# Autodesk Inventor assembly: EXTRUDER
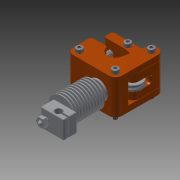
[picture p0: Inventor's stored thumbnail of the model, 180x180]
Saved by Autodesk Inventor 2013 (Build 170138000, 138)
## iProperties
Created: 2014-06-22
Part Number: EXTRUDER
Document SubType Name: Assembly
Designer: employee
Author: employee
## Documents named in this file (12)
- C:\Users\employee\Desktop\CoreXZ 2\EXTRUDER.iam
- C:\Users\employee\Desktop\CoreXZ 2\EXTRUDER BODY.ipt
- C:\Users\employee\Desktop\CoreXZ 2\E3Dv6.ipt
- C:\Users\employee\Desktop\CoreXZ 2\EXTRUDER BODY_MIR.ipt
- C:\Users\employee\Desktop\CoreXZ 2\EXTRUDER ARM.ipt
- C:\Users\employee\Desktop\CoreXZ 2\HOBBED PULLEY.ipt
- C:\Users\employee\Desktop\CoreXZ 2\625vv.ipt
- C:\Users\employee\Desktop\CoreXZ 2\EXTRUDER ARM_MIR.ipt
- C:\Users\employee\Desktop\CoreXZ 2\EXTRUDER SPRING.ipt
- C:\Users\employee\Desktop\CoreXZ 2\M3 SQUARE NUT.ipt
- C:\Users\employee\Desktop\CoreXZ 2\M3X35.ipt
- C:\Users\employee\Desktop\CoreXZ 2\M3X20.ipt
## Components (14 placed, 11 different names)
1. EXTRUDER BODY:1 — Insert:1, Angle:1, Flush:2, Insert:4, Angle:2, Insert:9
2. E3Dv6:1 — Insert:1, Angle:1
3. EXTRUDER BODY_MIR:1 — Mate:1, Insert:6, Insert:7, Insert:8
4. EXTRUDER ARM:1 — Insert:2, Insert:3, Flush:3, Insert:4, Mate:2, Flush:4
5. HOBBED PULLEY:1 — Mate:1, Flush:2
6. 625vv:1 — Insert:2
7. EXTRUDER ARM_MIR:1 — Insert:3, Flush:3, Insert:10
8. EXTRUDER SPRING:1 — Mate:2, Flush:4, Tangent:1, Mate:3, Mate:4
9. M3 SQUARE NUT:1 — Angle:2, Tangent:1, Mate:3
10. M3X35:1 — Insert:6
11. M3X35:2 — Insert:7
12. M3X35:3 — Insert:8
13. M3X35:4 — Insert:9, Mate:4
14. M3X20:1 — Insert:10
## Relationships (19: Insert 9, Mate 4, Flush 3, Angle 2, Tangent 1)
- Insert:1: EXTRUDER BODY:1 ↔ E3Dv6:1
- Angle:1 (0 deg): EXTRUDER BODY:1 ↔ E3Dv6:1
- Mate:1: EXTRUDER BODY_MIR:1 ↔ HOBBED PULLEY:1
- Flush:2 (7.38 mm): EXTRUDER BODY:1 ↔ HOBBED PULLEY:1
- Insert:2: EXTRUDER ARM:1 ↔ 625vv:1
- Insert:3: EXTRUDER ARM:1 ↔ EXTRUDER ARM_MIR:1
- Flush:3: EXTRUDER ARM:1 ↔ EXTRUDER ARM_MIR:1
- Insert:4: EXTRUDER BODY:1 ↔ EXTRUDER ARM:1
- Mate:2: EXTRUDER ARM:1 ↔ EXTRUDER SPRING:1
- Flush:4: EXTRUDER ARM:1 ↔ EXTRUDER SPRING:1
- Angle:2 (0 deg): EXTRUDER BODY:1 ↔ M3 SQUARE NUT:1
- Tangent:1: EXTRUDER SPRING:1 ↔ M3 SQUARE NUT:1
- Insert:6: EXTRUDER BODY_MIR:1 ↔ M3X35:1
- Insert:7: EXTRUDER BODY_MIR:1 ↔ M3X35:2
- Insert:8: EXTRUDER BODY_MIR:1 ↔ M3X35:3
- Mate:3: EXTRUDER SPRING:1 ↔ M3 SQUARE NUT:1
- Insert:9: EXTRUDER BODY:1 ↔ M3X35:4
- Mate:4: EXTRUDER SPRING:1 ↔ M3X35:4
- Insert:10: EXTRUDER ARM_MIR:1 ↔ M3X20:1
